# Autodesk Inventor assembly: Full payload assembly
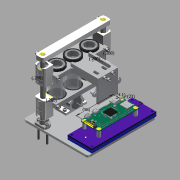
[picture p0: Inventor's stored thumbnail of the model, 180x180]
Saved by Autodesk Inventor 2017 (Build 210142000, 142)
## iProperties
Created: 2016-12-06
Part Number: Full payload assembly
Document SubType Name: Assembly
Designer: qupec
Author: qupec
## Documents named in this file (12)
- C:\Users\qupec\Desktop\UMD Near Space\STAR\CAD\Mechanical\Full payload assembly.iam
- C:\Users\qupec\Desktop\UMD Near Space\STAR\CAD\Mechanical\Base Plate.ipt
- C:\Users\qupec\Desktop\UMD Near Space\STAR\CAD\Mechanical\Slide rod assembly.iam
- C:\Users\qupec\Desktop\UMD Near Space\STAR\CAD\Mechanical\Test tube rack.iam
- C:\Users\qupec\Desktop\UMD Near Space\STAR\CAD\Mechanical\LED 5mm.ipt
- C:\Users\qupec\Desktop\UMD Near Space\STAR\CAD\Mechanical\STARduino and Pi assembly.iam
- C:\Users\qupec\Desktop\UMD Near Space\STAR\CAD\Mechanical\Pi Cam and Cable assembly.iam
- C:\Users\qupec\Desktop\UMD Near Space\STAR\CAD\Mechanical\Ribbon Cable Connector-02.ipt
- C:\Users\qupec\Desktop\UMD Near Space\RockSat\Full payload assembly\AIP\Cable and Harness\Full payload assembly.Harness2.iam
- C:\Users\qupec\Documents\Inventor\Content Center Files\R2017\en-US\U UNC 2603(1)\Unbrako - 4 x 1 - 48 - 1 - Unbrako.ipt
- C:\Users\qupec\Documents\Inventor\Content Center Files\R2017\en-US\ANSI B18.3(13)\ANSI B18.3 - 4-48 UNF - 0.625(22).ipt
- C:\Users\qupec\Desktop\UMD Near Space\STAR\CAD\Mechanical\ShakerCAD\ShakerAssembly.iam
## Components (23 placed, 11 different names)
1. Base Plate:1 — Flush:2, Flush:3, Flush:4, Mate:76, Mate:77, Mate:79, Flush:22, Flush:23, Mate:101, Flush:26, Flush:27, Mate:121, Mate:122, Mate:123
2. LED 5mm:1 — Mate:58, Mate:71, Mate:73, Mate:74
3. LED 5mm:2 — Mate:57, Mate:70, Mate:72, Mate:75
4. Slide rod assembly:1 [sub-assembly] — Mate:76, Mate:77, Mate:81, Mate:82, Mate:83, Mate:84, Mate:85, Mate:86, Mate:87, Mate:88, Mate:89, Mate:90, Mate:91, Mate:92, Mate:119, Mate:120, Flush:27
5. Test tube rack:1 [sub-assembly] — Mate:56, Flush:19, Flush:20, Mate:95, Mate:113, Mate:114, Mate:119, Mate:120
6. Pi Cam and Cable assembly:1 [sub-assembly] — Mate:56, Mate:57, Mate:58, Flush:19, Flush:20, Mate:70, Mate:71, Mate:72, Mate:73, Mate:74, Mate:75, Mate:93, Mate:94, Mate:96, Mate:97, Mate:98
7. Ribbon Cable Connector-02:1 — Mate:80, Flush:24, Flush:25
8. Harness2 [sub-assembly]
9. STARduino and Pi assembly:1 [sub-assembly] — Mate:79, Flush:22, Flush:23, Mate:80, Flush:24, Flush:25
10. Unbrako UNC Hex Socket Cap - Inch 4 x 1 - Unbrako:1 — Mate:82, Mate:91, Mate:123
11. Unbrako UNC Hex Socket Cap - Inch 4 x 1 - Unbrako:2 — Mate:81, Mate:90, Mate:122
12. Unbrako UNC Hex Socket Cap - Inch 4 x 1 - Unbrako:3 — Mate:83, Mate:92, Mate:121
13. Unbrako UNC Hex Socket Cap - Inch 4 x 1 - Unbrako:4 — Mate:85, Mate:87
14. Unbrako UNC Hex Socket Cap - Inch 4 x 1 - Unbrako:5 — Mate:84, Mate:89
15. Unbrako UNC Hex Socket Cap - Inch 4 x 1 - Unbrako:6 — Mate:86, Mate:88
16. Spline Socket Head Cap Screw - Inch 4-48 UNF - 0.625:1 — Mate:94, Mate:98
17. Spline Socket Head Cap Screw - Inch 4-48 UNF - 0.625:2 — Mate:95, Mate:96
18. Spline Socket Head Cap Screw - Inch 4-48 UNF - 0.625:3 — Mate:93, Mate:97
19. ShakerAssembly:1 [sub-assembly] — Mate:101, Mate:103, Mate:104, Mate:105, Mate:106, Mate:107, Mate:108, Mate:109, Mate:110, Mate:113, Mate:114, Flush:26
20. Unbrako UNC Hex Socket Cap - Inch 4 x 1 - Unbrako:7 — Mate:104, Mate:109
21. Unbrako UNC Hex Socket Cap - Inch 4 x 1 - Unbrako:8 — Mate:105, Mate:108
22. Unbrako UNC Hex Socket Cap - Inch 4 x 1 - Unbrako:9 — Mate:106, Mate:107
23. Unbrako UNC Hex Socket Cap - Inch 4 x 1 - Unbrako:10 — Mate:103, Mate:110
## Relationships (58: Mate 47, Flush 11)
- Flush:2: Base Plate:1
- Flush:3: Base Plate:1
- Flush:4: Base Plate:1
- Mate:56: Test tube rack:1 ↔ Pi Cam and Cable assembly:1
- Mate:57: LED 5mm:2 ↔ Pi Cam and Cable assembly:1
- Mate:58: LED 5mm:1 ↔ Pi Cam and Cable assembly:1
- Flush:19: Test tube rack:1 ↔ Pi Cam and Cable assembly:1
- Flush:20: Test tube rack:1 ↔ Pi Cam and Cable assembly:1
- Mate:70: LED 5mm:2 ↔ Pi Cam and Cable assembly:1
- Mate:71: LED 5mm:1 ↔ Pi Cam and Cable assembly:1
- Mate:72: LED 5mm:2 ↔ Pi Cam and Cable assembly:1
- Mate:73: LED 5mm:1 ↔ Pi Cam and Cable assembly:1
- Mate:74: LED 5mm:1 ↔ Pi Cam and Cable assembly:1
- Mate:75: LED 5mm:2 ↔ Pi Cam and Cable assembly:1
- Mate:76: Base Plate:1 ↔ Slide rod assembly:1
- Mate:77: Base Plate:1 ↔ Slide rod assembly:1
- Mate:79: Base Plate:1 ↔ STARduino and Pi assembly:1
- Flush:22: Base Plate:1 ↔ STARduino and Pi assembly:1
- Flush:23: Base Plate:1 ↔ STARduino and Pi assembly:1
- Mate:80: Ribbon Cable Connector-02:1 ↔ STARduino and Pi assembly:1
- Flush:24 (-7 mm): Ribbon Cable Connector-02:1 ↔ STARduino and Pi assembly:1
- Flush:25: Ribbon Cable Connector-02:1 ↔ STARduino and Pi assembly:1
- Mate:81: Slide rod assembly:1 ↔ Unbrako UNC Hex Socket Cap - Inch 4 x 1 - Unbrako:2
- Mate:82: Slide rod assembly:1 ↔ Unbrako UNC Hex Socket Cap - Inch 4 x 1 - Unbrako:1
- Mate:83: Slide rod assembly:1 ↔ Unbrako UNC Hex Socket Cap - Inch 4 x 1 - Unbrako:3
- Mate:84: Slide rod assembly:1 ↔ Unbrako UNC Hex Socket Cap - Inch 4 x 1 - Unbrako:5
- Mate:85: Slide rod assembly:1 ↔ Unbrako UNC Hex Socket Cap - Inch 4 x 1 - Unbrako:4
- Mate:86: Slide rod assembly:1 ↔ Unbrako UNC Hex Socket Cap - Inch 4 x 1 - Unbrako:6
- Mate:87: Slide rod assembly:1 ↔ Unbrako UNC Hex Socket Cap - Inch 4 x 1 - Unbrako:4
- Mate:88: Slide rod assembly:1 ↔ Unbrako UNC Hex Socket Cap - Inch 4 x 1 - Unbrako:6
- Mate:89: Slide rod assembly:1 ↔ Unbrako UNC Hex Socket Cap - Inch 4 x 1 - Unbrako:5
- Mate:90: Slide rod assembly:1 ↔ Unbrako UNC Hex Socket Cap - Inch 4 x 1 - Unbrako:2
- Mate:91: Slide rod assembly:1 ↔ Unbrako UNC Hex Socket Cap - Inch 4 x 1 - Unbrako:1
- Mate:92: Slide rod assembly:1 ↔ Unbrako UNC Hex Socket Cap - Inch 4 x 1 - Unbrako:3
- Mate:93: Pi Cam and Cable assembly:1 ↔ Spline Socket Head Cap Screw - Inch 4-48 UNF - 0.625:3
- Mate:94: Pi Cam and Cable assembly:1 ↔ Spline Socket Head Cap Screw - Inch 4-48 UNF - 0.625:1
- Mate:95: Test tube rack:1 ↔ Spline Socket Head Cap Screw - Inch 4-48 UNF - 0.625:2
- Mate:96: Pi Cam and Cable assembly:1 ↔ Spline Socket Head Cap Screw - Inch 4-48 UNF - 0.625:2
- Mate:97: Pi Cam and Cable assembly:1 ↔ Spline Socket Head Cap Screw - Inch 4-48 UNF - 0.625:3
- Mate:98: Pi Cam and Cable assembly:1 ↔ Spline Socket Head Cap Screw - Inch 4-48 UNF - 0.625:1
- Mate:101: Base Plate:1 ↔ ShakerAssembly:1
- Mate:103: ShakerAssembly:1 ↔ Unbrako UNC Hex Socket Cap - Inch 4 x 1 - Unbrako:10
- Mate:104: ShakerAssembly:1 ↔ Unbrako UNC Hex Socket Cap - Inch 4 x 1 - Unbrako:7
- Mate:105: ShakerAssembly:1 ↔ Unbrako UNC Hex Socket Cap - Inch 4 x 1 - Unbrako:8
- Mate:106: ShakerAssembly:1 ↔ Unbrako UNC Hex Socket Cap - Inch 4 x 1 - Unbrako:9
- Mate:107: ShakerAssembly:1 ↔ Unbrako UNC Hex Socket Cap - Inch 4 x 1 - Unbrako:9
- Mate:108: ShakerAssembly:1 ↔ Unbrako UNC Hex Socket Cap - Inch 4 x 1 - Unbrako:8
- Mate:109: ShakerAssembly:1 ↔ Unbrako UNC Hex Socket Cap - Inch 4 x 1 - Unbrako:7
- Mate:110: ShakerAssembly:1 ↔ Unbrako UNC Hex Socket Cap - Inch 4 x 1 - Unbrako:10
- Mate:113: Test tube rack:1 ↔ ShakerAssembly:1
- Mate:114: Test tube rack:1 ↔ ShakerAssembly:1
- Flush:26: Base Plate:1 ↔ ShakerAssembly:1
- Mate:119: Slide rod assembly:1 ↔ Test tube rack:1
- Mate:120: Slide rod assembly:1 ↔ Test tube rack:1
- Flush:27 (0.635 mm): Base Plate:1 ↔ Slide rod assembly:1
- Mate:121: Base Plate:1 ↔ Unbrako UNC Hex Socket Cap - Inch 4 x 1 - Unbrako:3
- Mate:122: Base Plate:1 ↔ Unbrako UNC Hex Socket Cap - Inch 4 x 1 - Unbrako:2
- Mate:123: Base Plate:1 ↔ Unbrako UNC Hex Socket Cap - Inch 4 x 1 - Unbrako:1
